# Autodesk Inventor assembly: Assembly
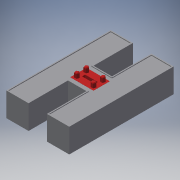
[picture p0: Inventor's stored thumbnail of the model, 180x180]
Saved by Autodesk Inventor 2018.3 (Build 223284000, 284)
## iProperties
Created: 2020-11-24
Part Number: Assembly
Document SubType Name: Assembly
Designer: daanv
Author: daanv
## Documents named in this file (3)
- C:\Users\daanv\OneDrive\Documenten\Life\Avans Project RED\Gebouw\Assembly.iam
- C:\Users\daanv\OneDrive\Documenten\Life\Avans Project RED\Gebouw\Gebouw Helix V1.ipt
- C:\Users\daanv\OneDrive\Documenten\Life\Avans Project RED\Gebouw\lego.ipt
## Components (2 placed, 2 different names)
1. Gebouw Helix V1:1 — Mate:1, Mate:2
2. lego:1 — Mate:1, Mate:2
## Relationships (2: Mate 2)
- Mate:1: Gebouw Helix V1:1 ↔ lego:1
- Mate:2: Gebouw Helix V1:1 ↔ lego:1
